# Autodesk Inventor assembly: Assembly1
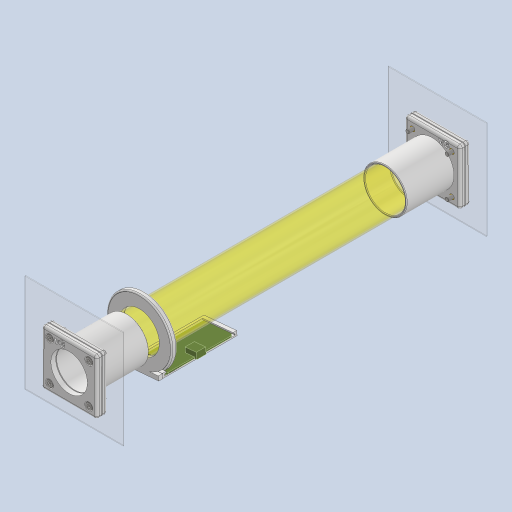
[picture p0: Inventor's stored thumbnail of the model, 512x512]
Saved by Autodesk Inventor 2024.4 (Build 284460000, 460)
## iProperties
Created: 2026-03-31
Part Number: Assembly1
Document SubType Name: Assembly
Designer: tooles01
Author: tooles01
## Documents named in this file (3)
- C:\Users\tooles01\NYU Langone Health Dropbox\Shannon Toole\Shannon_Dropbox\Mar lab\RFID\CAD\Cage_connector\Assembly1.iam
- C:\Users\tooles01\NYU Langone Health Dropbox\Shannon Toole\Shannon_Dropbox\Mar lab\RFID\CAD\Cage_connector\Cage_connector_v03.iam
- C:\Users\tooles01\NYU Langone Health Dropbox\Shannon Toole\Shannon_Dropbox\Mar lab\RFID\CAD\RFID_holder\RFID_holder_2piece.iam
## Components (3 placed, 2 different names)
1. Cage_connector_v03:1 [sub-assembly] — cage walls:spaced, cage walls flush:btm, cage walls flush:side, RFID_holder_to_tube:1, RFID_holder_to_tube:2
2. Cage_connector_v03:2 [sub-assembly] — cage walls:spaced, cage walls flush:btm, cage walls flush:side
3. RFID_holder_2piece:1 [sub-assembly] — RFID_holder_to_tube:1, RFID_holder_to_tube:2
## Relationships (5: Mate 3, Flush 2)
- cage walls:spaced [Mate] (295.275 mm): Cage_connector_v03:1 ↔ Cage_connector_v03:2
- cage walls flush:btm [Flush]: Cage_connector_v03:1 ↔ Cage_connector_v03:2
- cage walls flush:side [Flush]: Cage_connector_v03:1 ↔ Cage_connector_v03:2
- RFID_holder_to_tube:1 [Mate]: Cage_connector_v03:1 ↔ RFID_holder_2piece:1
- RFID_holder_to_tube:2 [Mate] (10 mm): Cage_connector_v03:1 ↔ RFID_holder_2piece:1
